# Autodesk Inventor assembly: 30mm
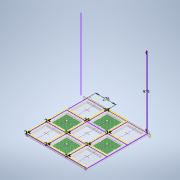
[picture p0: Inventor's stored thumbnail of the model, 180x180]
Saved by Autodesk Inventor 2021 (Build 250183000, 183)
## iProperties
Created: 2020-11-09
Part Number: 30mm
Document SubType Name: Assembly
Designer: Wes
_SolveAssemblyDoc: Frame Generator Solve Assembly
_Version: 25.0.0
Author: Wes
## Documents named in this file (6)
- C:\Users\Wes\Dropbox\8020 DDR Pad\30mm.iam
- C:\Users\Wes\Dropbox\8020 DDR Pad\Part1.ipt
- C:\Users\Wes\Dropbox\8020 DDR Pad\30mm\Frame\Frame 1604985372804.iam
- C:\Users\Wes\Dropbox\8020 DDR Pad\Arrow Panel.ipt
- C:\Users\Wes\Documents\Inventor\Content Center Files\R2021\en-US\ISO 4762(2)\ISO 4762 - M5 x 16ISO.ipt
- C:\Users\Wes\Dropbox\DDR Pad\DDR Pad\DDR Pad 1.ipt
## Components (16 placed, 5 different names)
1. Part1:1 — Planar:1, Planar:2, Planar:3, Planar:4, Planar:5, Planar:6, Planar:7, Planar:8, Planar:9, Rigid:1, Rigid:2, Rigid:3, Rigid:4, Mate:3
2. Frame 1604985372804:1 [sub-assembly] — Angle:1
3. Arrow Panel:1 — Mate:1, Mate:2, Planar:5
4. Arrow Panel:2 — Planar:6
5. Arrow Panel:3 — Planar:8
6. Arrow Panel:4 — Planar:9
7. Arrow Panel:5 — Planar:7
8. Arrow Panel:6 — Planar:4
9. Arrow Panel:7 — Planar:3
10. Arrow Panel:8 — Planar:2
11. Arrow Panel:9 — Planar:1
12. ISO 4762 M5 x 16:1 — Mate:1, Mate:2
13. DDR Pad 1:1 — Rigid:1
14. DDR Pad 1:2 — Rigid:4
15. DDR Pad 1:3 — Rigid:2
16. DDR Pad 1:4 — Rigid:3
## Relationships (17: PlanarJoint 9, WeldJoint 4, Mate 3, Angle 1)
- Mate:1: Arrow Panel:1 ↔ ISO 4762 M5 x 16:1
- Mate:2: Arrow Panel:1 ↔ ISO 4762 M5 x 16:1
- Planar:1: Part1:1 ↔ Arrow Panel:9
- Planar:2: Part1:1 ↔ Arrow Panel:8
- Planar:3: Part1:1 ↔ Arrow Panel:7
- Planar:4: Part1:1 ↔ Arrow Panel:6
- Planar:5: Part1:1 ↔ Arrow Panel:1
- Planar:6: Part1:1 ↔ Arrow Panel:2
- Planar:7: Part1:1 ↔ Arrow Panel:5
- Planar:8: Part1:1 ↔ Arrow Panel:3
- Planar:9: Part1:1 ↔ Arrow Panel:4
- Rigid:1 [WeldJoint] (-15 mm): Part1:1 ↔ DDR Pad 1:1
- Rigid:2 [WeldJoint] (-15 mm): Part1:1 ↔ DDR Pad 1:3
- Rigid:3 [WeldJoint] (-15 mm): Part1:1 ↔ DDR Pad 1:4
- Rigid:4 [WeldJoint] (-15 mm): Part1:1 ↔ DDR Pad 1:2
- Mate:3: Part1:1
- Angle:1 (0 deg): Frame 1604985372804:1
